# Autodesk Inventor assembly: 出力板ユニット
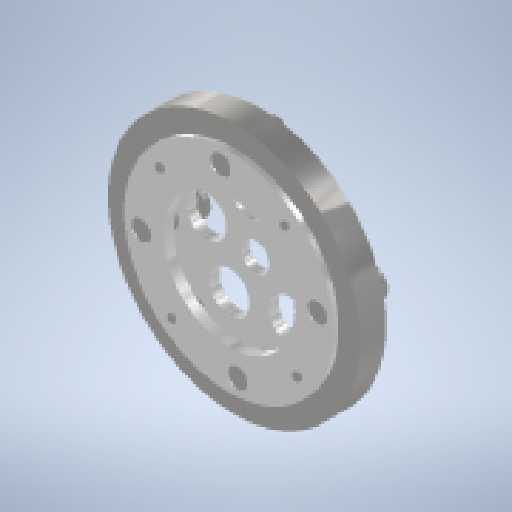
[picture p0: Inventor's stored thumbnail of the model, 512x512]
Saved by Autodesk Inventor 2024 (Build 280153000, 153)
## iProperties
Created: 2023-05-29
Part Number: 出力板ユニット
Document SubType Name: Assembly
Designer: yuta2
Mass: 503.335 g
Surface Area: 553.016 cm^2
Volume: 117.857 cm^3
Density: 4.27073 g/cm^3
Author: yuta2
## Documents named in this file (18)
- C:\Users\yuta2\Documents\Inventor\CycloidDrive\サイクロイド減速機_大型\出力板ユニット.iam
- C:\Users\yuta2\Documents\Inventor\CycloidDrive\ベアリング\6820ZZ.ipt
- C:\Users\yuta2\Documents\Inventor\CycloidDrive\サイクロイド減速機_大型\出力板.ipt
- C:\Users\yuta2\Documents\Inventor\CycloidDrive\サイクロイド減速機_大型\出力板表.ipt
- C:\Users\yuta2\Documents\Inventor\CycloidDrive\サイクロイド減速機_大型\出力ピンユニット.iam
- C:\Users\yuta2\Documents\Inventor\CycloidDrive\サイクロイド減速機_大型\出力板ユニット\デザイン アクセラレータ\ボルト締結1.iam
- C:\Users\yuta2\Documents\Inventor\CycloidDrive\サイクロイド減速機_大型\出力板ユニット\AIP\FEA\ecnbbtdpc.fins
- C:\Users\yuta2\Documents\Inventor\CycloidDrive\サイクロイド減速機_大型\出力板ユニット\AIP\FEA\ecnbbtdq8.fsat
- C:\Users\yuta2\Documents\Inventor\CycloidDrive\サイクロイド減速機_大型\出力板ユニット\AIP\FEA\ecnbbtdq8.ftes
- C:\Users\yuta2\Documents\Inventor\CycloidDrive\サイクロイド減速機_大型\出力板ユニット\AIP\FEA\ecnbbtdq8.fwiz
- C:\Users\yuta2\Documents\Inventor\CycloidDrive\サイクロイド減速機_大型\出力板ユニット\AIP\FEA\ecnbbtds0.fmsh
- C:\Users\yuta2\Documents\Inventor\CycloidDrive\サイクロイド減速機_大型\出力板ユニット\AIP\FEA\ecnbbtdsw.fres
- C:\Users\yuta2\Documents\Inventor\CycloidDrive\サイクロイド減速機_大型\出力板ユニット\AIP\FEA\ecocrey3k.fins
- C:\Users\yuta2\Documents\Inventor\CycloidDrive\サイクロイド減速機_大型\出力板ユニット\AIP\FEA\ecocrey3k.fsat
- C:\Users\yuta2\Documents\Inventor\CycloidDrive\サイクロイド減速機_大型\出力板ユニット\AIP\FEA\ecocrey3k.ftes
- C:\Users\yuta2\Documents\Inventor\CycloidDrive\サイクロイド減速機_大型\出力板ユニット\AIP\FEA\ecocrey3k.fwiz
- C:\Users\yuta2\Documents\Inventor\CycloidDrive\サイクロイド減速機_大型\出力板ユニット\AIP\FEA\ecocreybk.fmsh
- C:\Users\yuta2\Documents\Inventor\CycloidDrive\サイクロイド減速機_大型\出力板ユニット\AIP\FEA\ecocreybl.fres
## Components (11 placed, 5 different names)
1. 6820ZZ:1 — 回転:1, 回転:3
2. 出力板:1 — 回転:1, 回転:4, メイト:1, メイト:2
3. 出力板表:1 — 回転:3, 円柱状:1
4. 出力ピンユニット:1 [sub-assembly] — 回転:4, 円柱状:1
5. 出力ピンユニット:2 [sub-assembly]
6. 出力ピンユニット:3 [sub-assembly]
7. 出力ピンユニット:4 [sub-assembly]
8. ボルト締結:1 [sub-assembly] — メイト:1, メイト:2
9. ボルト締結:2 [sub-assembly]
10. ボルト締結:3 [sub-assembly]
11. ボルト締結:4 [sub-assembly]
## Component patterns: (4 elements, first: 出力ピンユニット:1), (4 elements, first: ボルト締結:1)
## Relationships (6: RevoluteJoint 3, Mate 2, CylindricalJoint 1)
- 回転:1 [RevoluteJoint]: 6820ZZ:1 ↔ 出力板:1
- 回転:3 [RevoluteJoint]: 6820ZZ:1 ↔ 出力板表:1
- 回転:4 [RevoluteJoint]: 出力板:1 ↔ 出力ピンユニット:1
- 円柱状:1 [CylindricalJoint]: 出力板表:1 ↔ 出力ピンユニット:1
- メイト:1 [Mate]: 出力板:1 ↔ ボルト締結:1
- メイト:2 [Mate]: 出力板:1 ↔ ボルト締結:1
## Named parameters: sa_0 = 100000, sa_1 = 500000, sa_2 = 500000
note: some values were not read from the file. Shown as the stored number, unit unknown: "sa_0", "sa_1", "sa_2".
